# Autodesk Inventor assembly: 5 Barras Version 0
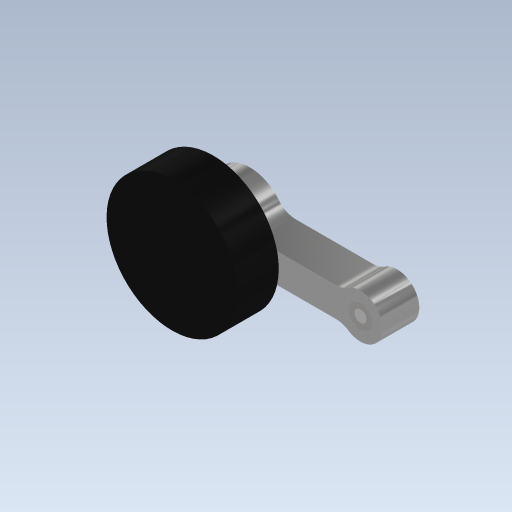
[picture p0: Inventor's stored thumbnail of the model, 512x512]
Saved by Autodesk Inventor 2024.2 (Build 282272000, 272)
## iProperties
Created: 2025-02-06
Part Number: 5 Barras Version 0
Document SubType Name: Assembly
Designer: jp.reyesf
Author: jp.reyesf
## Documents named in this file (8)
- C:\Users\jp.reyesf\Desktop\Master-Thesis\five_bar\assets\CAD\Robot\Subassemblies\Proximal Link 1.iam
- C:\Users\jp.reyesf\Desktop\Master-Thesis\five_bar\assets\CAD\Robot\Proximal Link 2.ipt
- C:\Users\jp.reyesf\Desktop\Master-Thesis\five_bar\assets\CAD\Robot\Spacer.ipt
- C:\Users\jp.reyesf\Desktop\Master-Thesis\five_bar\assets\CAD\Robot\Bearing.ipt
- C:\Users\jp.reyesf\Desktop\Master-Thesis\five_bar\assets\CAD\Robot\Motor 2 Rotor.ipt
- C:\Users\jp.reyesf\Desktop\Master-Thesis\five_bar\assets\CAD\Robot\separator.ipt
- C:\Users\jp.reyesf\Desktop\Master-Thesis\five_bar\assets\CAD\Robot\rod.ipt
- C:\Users\jp.reyesf\Desktop\Master-Thesis\five_bar\assets\CAD\Robot\Subassemblies\DummyBar.ipt
## Components (8 placed, 7 different names)
1. Proximal Link 2:1 — Mate:35, Flush:6, Mate:48, Mate:49, Flush:9, Mate:54, Mate:55, Flush:10, Angle:1, Mate:58, Flush:11
2. Motor 2 Rotor:1 — Mate:48, Mate:49, Mate:55, Mate:57
3. separator:2 — Mate:56, Mate:58
4. Spacer:2 — Mate:35
5. Bearing:4 — Flush:6, Mate:59
6. Bearing:5
7. rod:3 — Flush:9, Mate:54, Mate:56
8. DummyBar:1 — Mate:59, Flush:11
## Relationships (18: Mate 13, Flush 4, Angle 1)
- [Mate]: Spacer:2 ↔ Bearing:4
- [Mate]: Spacer:2 ↔ Bearing:5
- [Mate]: Spacer:2 ↔ Bearing:4
- [Mate]: Spacer:2 ↔ Bearing:5
- Mate:35: Proximal Link 2:1 ↔ Spacer:2
- Flush:6: Proximal Link 2:1 ↔ Bearing:4
- Mate:48: Proximal Link 2:1 ↔ Motor 2 Rotor:1
- Mate:49: Proximal Link 2:1 ↔ Motor 2 Rotor:1
- Flush:9: Proximal Link 2:1 ↔ rod:3
- Mate:54: Proximal Link 2:1 ↔ rod:3
- Mate:55: Proximal Link 2:1 ↔ Motor 2 Rotor:1
- Mate:56: separator:2 ↔ rod:3
- Mate:57: Motor 2 Rotor:1
- Flush:10: Proximal Link 2:1
- Angle:1 (180 deg): Proximal Link 2:1
- Mate:58: Proximal Link 2:1 ↔ separator:2
- Mate:59: Bearing:4 ↔ DummyBar:1
- Flush:11: Proximal Link 2:1 ↔ DummyBar:1
## Named parameters: d18_d14 = 0 mm, d19_d15 = 0 mm, d20_d16 = 0 mm, d21_d17 = 0 mm
